# Autodesk Inventor assembly: BHSS
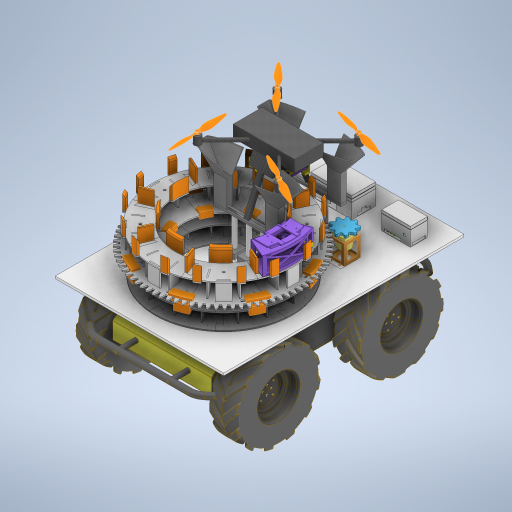
[picture p0: Inventor's stored thumbnail of the model, 512x512]
Saved by Autodesk Inventor 2023 (Build 270158000, 158)
## iProperties
Created: 2022-10-26
Part Number: BHSS
Document SubType Name: Assembly
Designer: cheng
Mass: 18338.5 g
Surface Area: 54431.4 cm^2
Volume: 16113.2 cm^3
Density: 1.1381 g/cm^3
Author: cheng
## Documents named in this file (14)
- C:\Users\mihal\Desktop\4th Year Project\Final Assembly\BHSS.iam
- C:\Users\mihal\Desktop\4th Year Project\Final Assembly\Drone_Model.ipt
- C:\Users\mihal\Desktop\4th Year Project\Final Assembly\Husky_3D_Model.ipt
- C:\Users\mihal\Desktop\4th Year Project\Final Assembly\Rotating Carousel\Moving Carousel Assembly.iam
- C:\Users\mihal\Desktop\4th Year Project\Final Assembly\Non-Rotating Carousel\Non-Rotating Carousel Assembly.iam
- C:\Users\mihal\Desktop\4th Year Project\Final Assembly\Battery Cage and Sprind Plate\Battery Cage Assembly.iam
- C:\Users\mihal\Desktop\4th Year Project\Final Assembly\Motor Casing\Motor Assembly.iam
- C:\Users\mihal\Desktop\4th Year Project\Final Assembly\Base Plate\Base Plate.ipt
- C:\Users\mihal\Desktop\4th Year Project\Final Assembly\Battery Module\Battery Module.iam
- C:\Users\mihal\Desktop\4th Year Project\Final Assembly\Landing Docks\Landing Docks Assembly.iam
- C:\Users\mihal\Desktop\4th Year Project\Final Assembly\Motor Casing\Motor Gear.ipt
- C:\Users\mihal\Desktop\4th Year Project\Final Assembly\Propeller 10x45.ipt
- C:\Users\mihal\Desktop\4th Year Project\Final Assembly\Power Supply Box\Power Supply Box.iam
- C:\Users\mihal\Desktop\4th Year Project\Final Assembly\Board Box\Board Box.iam
## Components (17 placed, 13 different names)
1. Drone_Model:1 — Mate:129, Mate:130, Mate:131, Mate:145, Mate:146, Mate:147, Flush:6, Mate:164, Mate:165, Mate:166, Mate:167, Mate:168, Mate:169, Mate:170, Mate:171, Mate:175
2. Husky_3D_Model:1 — Flush:5, Mate:148, Mate:149
3. Moving Carousel Assembly:1 [sub-assembly] — Mate:117, Mate:118, ROTATION CONSTRAINT, Mate:139, Angle:4, Mate:172
4. Non-Rotating Carousel Assembly:1 [sub-assembly] — Mate:117, Mate:118, ROTATION CONSTRAINT, Mate:150, Mate:157, Mate:158
5. Base Plate:1 — Flush:5, Mate:148, Mate:149, Mate:150, Mate:151, Mate:152, Mate:153, Mate:154, Mate:157, Mate:158, Mate:160, Mate:161, Mate:162, Mate:173, Mate:174, Mate:177, Mate:178
6. Battery Cage Assembly:1 [sub-assembly] — Mate:129, Mate:130, Mate:131, Mate:145, Mate:146, Mate:147
7. Motor Gear:1
8. Motor Assembly:1 [sub-assembly] — Mate:160, Mate:161, Mate:162
9. Landing Docks Assembly:1 [sub-assembly] — Mate:151, Mate:153, Flush:6, Mate:173, Mate:175
10. Landing Docks Assembly:2 [sub-assembly] — Mate:152, Mate:154, Mate:174
11. Battery Module:6 [sub-assembly] — Mate:139, Angle:4, Mate:172
12. Propeller 10x45:1 — Mate:166, Mate:167
13. Propeller 10x45:2 — Mate:170, Mate:171
14. Propeller 10x45:3 — Mate:164, Mate:165
15. Propeller 10x45:4 — Mate:168, Mate:169
16. Power Supply Box:1 [sub-assembly] — Mate:177
17. Board Box:1 [sub-assembly] — Mate:178
## Relationships (41: Mate 36, Flush 3, Angle 2)
- Mate:117: Moving Carousel Assembly:1 ↔ Non-Rotating Carousel Assembly:1
- Mate:118: Moving Carousel Assembly:1 ↔ Non-Rotating Carousel Assembly:1
- Mate:129: Drone_Model:1 ↔ Battery Cage Assembly:1
- Mate:130: Drone_Model:1 ↔ Battery Cage Assembly:1
- Mate:131: Drone_Model:1 ↔ Battery Cage Assembly:1
- ROTATION CONSTRAINT [Angle] (60 deg): Moving Carousel Assembly:1 ↔ Non-Rotating Carousel Assembly:1
- Mate:139: Moving Carousel Assembly:1 ↔ Battery Module:6
- Angle:4 (180 deg): Moving Carousel Assembly:1 ↔ Battery Module:6
- Mate:145: Drone_Model:1 ↔ Battery Cage Assembly:1
- Mate:146: Drone_Model:1 ↔ Battery Cage Assembly:1
- Mate:147: Drone_Model:1 ↔ Battery Cage Assembly:1
- Flush:5: Husky_3D_Model:1 ↔ Base Plate:1
- Mate:148: Husky_3D_Model:1 ↔ Base Plate:1
- Mate:149: Husky_3D_Model:1 ↔ Base Plate:1
- Mate:150: Non-Rotating Carousel Assembly:1 ↔ Base Plate:1
- Mate:151: Base Plate:1 ↔ Landing Docks Assembly:1
- Mate:152: Base Plate:1 ↔ Landing Docks Assembly:2
- Mate:153: Base Plate:1 ↔ Landing Docks Assembly:1
- Mate:154: Base Plate:1 ↔ Landing Docks Assembly:2
- Mate:157: Non-Rotating Carousel Assembly:1 ↔ Base Plate:1
- Mate:158: Non-Rotating Carousel Assembly:1 ↔ Base Plate:1
- Flush:6: Drone_Model:1 ↔ Landing Docks Assembly:1
- Mate:160: Base Plate:1 ↔ Motor Assembly:1
- Mate:161: Base Plate:1 ↔ Motor Assembly:1
- Mate:162: Base Plate:1 ↔ Motor Assembly:1
- [Mate]: Motor Gear:1 ↔ Motor Assembly:1
- [Flush]: Motor Gear:1 ↔ Motor Assembly:1
- Mate:164: Drone_Model:1 ↔ Propeller 10x45:3
- Mate:165: Drone_Model:1 ↔ Propeller 10x45:3
- Mate:166: Drone_Model:1 ↔ Propeller 10x45:1
- Mate:167: Drone_Model:1 ↔ Propeller 10x45:1
- Mate:168: Drone_Model:1 ↔ Propeller 10x45:4
- Mate:169: Drone_Model:1 ↔ Propeller 10x45:4
- Mate:170: Drone_Model:1 ↔ Propeller 10x45:2
- Mate:171: Drone_Model:1 ↔ Propeller 10x45:2
- Mate:172: Moving Carousel Assembly:1 ↔ Battery Module:6
- Mate:173: Base Plate:1 ↔ Landing Docks Assembly:1
- Mate:174: Base Plate:1 ↔ Landing Docks Assembly:2
- Mate:175: Drone_Model:1 ↔ Landing Docks Assembly:1
- Mate:177: Base Plate:1 ↔ Power Supply Box:1
- Mate:178: Base Plate:1 ↔ Board Box:1
